# Autodesk Inventor assembly: pneumatic area
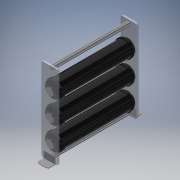
[picture p0: Inventor's stored thumbnail of the model, 180x180]
Saved by Autodesk Inventor 2019 (Build 230136000, 136)
## iProperties
Created: 2019-02-02
Part Number: pneumatic area
Document SubType Name: Assembly
Designer: rachala.rohit
Author: rachala.rohit
## Documents named in this file (5)
- \\fs1\studentusers\class22\Rachala.Rohit\documents\Laptop Inventor\2019Robot\pneumatic area.iam
- \\fs1\studentusers\class22\Rachala.Rohit\documents\Laptop Inventor\2019Robot\t slot bar.ipt
- \\fs1\studentusers\class22\Rachala.Rohit\documents\Laptop Inventor\2019Robot\plate for pneumatic holder.ipt
- \\fs1\studentusers\class22\Rachala.Rohit\documents\Laptop Inventor\2019Robot\holder.ipt
- \\fs1\studentusers\class22\Rachala.Rohit\documents\Laptop Inventor\2019Robot\clippard pneumatic.ipt
## Components (9 placed, 4 different names)
1. t slot bar:1 — Mate:7, Mate:8, Mate:9
2. plate for pneumatic holder:1 — Mate:4, Mate:5, Mate:6, Mate:7, Mate:8, Mate:9, Mate:10, Mate:12, Mate:13, Mate:14, Mate:15, Mate:16, Mate:17, Mate:18, Mate:19
3. holder:1 — Mate:23, Mate:24, Mate:25
4. holder:2 — Mate:4, Mate:5, Mate:6
5. t slot bar:2 — Mate:10, Mate:12, Mate:19, Mate:20, Mate:21, Mate:22
6. clippard pneumatic:1 — Mate:17, Mate:18
7. clippard pneumatic:2 — Mate:13, Mate:14
8. clippard pneumatic:3 — Mate:15, Mate:16
9. plate for pneumatic holder:2 — Mate:20, Mate:21, Mate:22, Mate:23, Mate:24, Mate:25
## Relationships (21: Mate 21)
- Mate:4: plate for pneumatic holder:1 ↔ holder:2
- Mate:5 (-27.432 mm): plate for pneumatic holder:1 ↔ holder:2
- Mate:6 (-54.229 mm): plate for pneumatic holder:1 ↔ holder:2
- Mate:7: t slot bar:1 ↔ plate for pneumatic holder:1
- Mate:8 (-19.05 mm): t slot bar:1 ↔ plate for pneumatic holder:1
- Mate:9 (-38.1 mm): t slot bar:1 ↔ plate for pneumatic holder:1
- Mate:10 (-19.05 mm): plate for pneumatic holder:1 ↔ t slot bar:2
- Mate:12 (-38.1 mm): plate for pneumatic holder:1 ↔ t slot bar:2
- Mate:13: plate for pneumatic holder:1 ↔ clippard pneumatic:2
- Mate:14 (-6.35 mm): plate for pneumatic holder:1 ↔ clippard pneumatic:2
- Mate:15: plate for pneumatic holder:1 ↔ clippard pneumatic:3
- Mate:16 (-6.35 mm): plate for pneumatic holder:1 ↔ clippard pneumatic:3
- Mate:17: plate for pneumatic holder:1 ↔ clippard pneumatic:1
- Mate:18 (-6.35 mm): plate for pneumatic holder:1 ↔ clippard pneumatic:1
- Mate:19: plate for pneumatic holder:1 ↔ t slot bar:2
- Mate:20: t slot bar:2 ↔ plate for pneumatic holder:2
- Mate:21 (-19.05 mm): t slot bar:2 ↔ plate for pneumatic holder:2
- Mate:22 (-38.1 mm): t slot bar:2 ↔ plate for pneumatic holder:2
- Mate:23 (-27.432 mm): holder:1 ↔ plate for pneumatic holder:2
- Mate:24: holder:1 ↔ plate for pneumatic holder:2
- Mate:25 (-54.229 mm): holder:1 ↔ plate for pneumatic holder:2
